# Autodesk Inventor assembly: Elevator
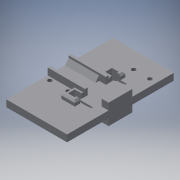
[picture p0: Inventor's stored thumbnail of the model, 180x180]
Saved by Autodesk Inventor 2016 (Build 200138000, 138)
## iProperties
Created: 2017-10-26
Part Number: Elevator
Document SubType Name: Assembly
Designer: thompson.nathaniel
Author: thompson.nathaniel
## Documents named in this file (3)
- \\fs1\studentusers\class18\Thompson.Nathaniel\Documents\Engineering\Elevator.iam
- \\fs1\studentusers\class18\Thompson.Nathaniel\Documents\Engineering\Elevator Slide Top.ipt
- \\fs1\studentusers\class18\Thompson.Nathaniel\Documents\Engineering\Elevator Slide.ipt
## Components (2 placed, 2 different names)
1. Elevator Slide Top:1 — Flush:1, Flush:2, Mate:1
2. Elevator Slide:1 — Flush:1, Flush:2, Mate:1
## Relationships (3: Flush 2, Mate 1)
- Flush:1: Elevator Slide Top:1 ↔ Elevator Slide:1
- Flush:2: Elevator Slide Top:1 ↔ Elevator Slide:1
- Mate:1: Elevator Slide Top:1 ↔ Elevator Slide:1
